# Autodesk Inventor assembly: AssemblyFullPrinter
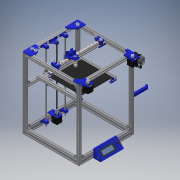
[picture p0: Inventor's stored thumbnail of the model, 180x180]
Saved by Autodesk Inventor 2018 (Build 220112000, 112)
## iProperties
Created: 2017-10-01
Part Number: AssemblyFullPrinter
Document SubType Name: Assembly
Designer: Jurjen
Author: Jurjen
## Documents named in this file (51)
- C:\Users\Jurjen\Documents\3D Printer\coreXY\Mechanical\AssemblyFullPrinter.iam
- C:\Users\Jurjen\Documents\3D Printer\coreXY\Mechanical\2020-350mm.ipt
- C:\Users\Jurjen\Documents\3D Printer\coreXY\Mechanical\2020-500mm.ipt
- C:\Users\Jurjen\Documents\3D Printer\coreXY\Mechanical\2020-corner-bracket.ipt
- C:\Users\Jurjen\Documents\3D Printer\coreXY\Mechanical\heated-bed.ipt
- C:\Users\Jurjen\Documents\3D Printer\coreXY\Mechanical\T8-lead-screw.ipt
- C:\Users\Jurjen\Documents\3D Printer\coreXY\Mechanical\motedis\GT2-Pulley-20-Teeth-5mm-Bore.ipt
- C:\Users\Jurjen\Documents\3D Printer\coreXY\Mechanical\motedis\Gt20.ipt
- C:\Users\Jurjen\Documents\3D Printer\coreXY\Mechanical\motedis\shaft-couple-flex.ipt
- C:\Users\Jurjen\Documents\3D Printer\coreXY\Mechanical\rod-8mm.ipt
- C:\Users\Jurjen\Documents\3D Printer\coreXY\Mechanical\2020-290mm.ipt
- C:\Users\Jurjen\Documents\3D Printer\coreXY\Mechanical\2020-240mm.ipt
- C:\Users\Jurjen\Documents\3D Printer\coreXY\Mechanical\T8x2mm lead screw.ipt
- C:\Users\Jurjen\Documents\3D Printer\coreXY\Mechanical\OldhamCouplerBottom.ipt
- C:\Users\Jurjen\Documents\3D Printer\coreXY\Mechanical\OldhamCouplerMiddle.ipt
- C:\Users\Jurjen\Documents\3D Printer\coreXY\Mechanical\OldhamCouplerTop.ipt
- C:\Users\Jurjen\Documents\3D Printer\coreXY\Mechanical\M5-nut.ipt
- C:\Users\Jurjen\Documents\3D Printer\coreXY\Mechanical\bracket-GT2-left.ipt
- C:\Users\Jurjen\Documents\3D Printer\coreXY\Mechanical\M5x30mm.ipt
- C:\Users\Jurjen\Documents\3D Printer\coreXY\Mechanical\mount-heated-bed.ipt
- C:\Users\Jurjen\Documents\3D Printer\coreXY\Mechanical\bracket-GT2-right.ipt
- C:\Users\Jurjen\Documents\3D Printer\coreXY\Mechanical\spool-holder.ipt
- C:\Users\Jurjen\Documents\3D Printer\coreXY\Mechanical\nema-17.ipt
- C:\Users\Jurjen\Documents\3D Printer\coreXY\Mechanical\nema17-mount-left.ipt
- C:\Users\Jurjen\Documents\3D Printer\coreXY\Mechanical\nema17-mount-right.ipt
- C:\Users\Jurjen\Documents\3D Printer\coreXY\Mechanical\LMF8LUU.ipt
- C:\Users\Jurjen\Documents\3D Printer\coreXY\Mechanical\MGN-12-rail.ipt
- C:\Users\Jurjen\Documents\3D Printer\coreXY\Mechanical\2020-320mm.ipt
- C:\Users\Jurjen\Documents\3D Printer\coreXY\Mechanical\x-carriage-2020.ipt
- C:\Users\Jurjen\Documents\3D Printer\coreXY\Mechanical\X-connector-left.ipt
- C:\Users\Jurjen\Documents\3D Printer\coreXY\Mechanical\X-connector-right.ipt
- C:\Users\Jurjen\Documents\3D Printer\coreXY\Mechanical\MGN-12-H-carriage.ipt
- C:\Users\Jurjen\Documents\3D Printer\coreXY\Mechanical\ED3V6.ipt
- C:\Users\Jurjen\Documents\3D Printer\coreXY\Mechanical\x-carriage.ipt
- C:\Users\Jurjen\Documents\3D Printer\coreXY\Mechanical\x-carriage-holder.ipt
- C:\Users\Jurjen\Documents\3D Printer\coreXY\Mechanical\holder-GT2-x-carriage-left.ipt
- C:\Users\Jurjen\Documents\3D Printer\coreXY\Mechanical\M5x35mm-crosshead.ipt
- C:\Users\Jurjen\Documents\3D Printer\coreXY\Mechanical\extruder\e3d titan.iam
- C:\Users\Jurjen\Documents\3D Printer\coreXY\Mechanical\mount-extruder.ipt
- C:\Users\Jurjen\Documents\3D Printer\coreXY\Mechanical\NylonSpacerM5x5mm.ipt
- C:\Users\Jurjen\Documents\3D Printer\coreXY\Mechanical\holder-GT2-x-carriage-right.ipt
- C:\Users\Jurjen\Documents\3D Printer\coreXY\Mechanical\holder-bearing-z-axis.ipt
- C:\Users\Jurjen\Documents\3D Printer\coreXY\Mechanical\2040-350mm.ipt
- C:\Users\Jurjen\Documents\3D Printer\coreXY\Mechanical\nema17-mount-bottom-z-axis-v2.ipt
- C:\Users\Jurjen\Documents\3D Printer\coreXY\Mechanical\ramps-1.4 2004-LCD.ipt
- C:\Users\Jurjen\Documents\3D Printer\coreXY\Mechanical\holder-LCD-screen.ipt
- C:\Users\Jurjen\Documents\3D Printer\coreXY\Mechanical\spring-25mm.ipt
- C:\Users\Jurjen\Documents\3D Printer\coreXY\Mechanical\M3x40mm.ipt
- C:\Users\Jurjen\Documents\3D Printer\coreXY\Mechanical\2040-360mm.ipt
- C:\Users\Jurjen\Documents\3D Printer\coreXY\Mechanical\SH8.ipt
- C:\Users\Jurjen\Documents\3D Printer\coreXY\Mechanical\holder-LMF8LUU-z-axis-v2.ipt
## Components (135 placed, 50 different names)
1. SH8:1 — Mate:601, Mate:602, Mate:603, Mate:604
2. SH8:2 — Mate:598, Mate:599, Mate:600, Mate:605
3. SH8:3 — Mate:606, Mate:607, Mate:611
4. SH8:4 — Mate:608, Mate:609, Mate:610
5. holder-LMF8LUU-z-axis-v2:1 — Mate:612, Mate:613, Mate:614, Mate:615, Mate:616, Mate:623
6. holder-LMF8LUU-z-axis-v2:2 — Mate:617, Mate:619, Mate:620, Mate:621, Mate:622
7. 2020-500mm:1 — Mate:1, Flush:2, Flush:14, Mate:90, Mate:92, Mate:93, Mate:94, Mate:166, Mate:168, Mate:287, Mate:288, Flush:54, Mate:359, Mate:360, Mate:459, Mate:471, Mate:472, Mate:473, Flush:92, Mate:552, Flush:107
8. 2020-500mm:2 — Mate:2, Flush:1, Flush:13, Flush:14, Mate:75, Mate:77, Mate:79, Mate:80, Mate:151, Mate:152, Mate:362, Mate:455, Mate:530, Flush:93, Mate:563, Flush:109, Flush:110
9. 2020-500mm:3 — Mate:8, Flush:12, Flush:13, Flush:15, Mate:82, Mate:83, Mate:136, Mate:138, Flush:67, Mate:367, Mate:456, Mate:501, Flush:85, Flush:86, Mate:516, Mate:517, Mate:562, Mate:585, Mate:591, Flush:115
10. 2020-500mm:4 — Mate:7, Flush:15, Flush:27, Mate:142, Mate:144, Mate:157, Mate:158, Mate:354, Flush:65, Mate:447, Mate:450, Mate:510, Mate:553, Flush:106, Mate:575, Flush:114, Mate:583, Mate:596
11. 2020-corner-bracket:38 — Mate:515, Mate:516, Mate:517
12. 2020-320mm:3 — Mate:353, Mate:354, Mate:355, Mate:356, Flush:65, Flush:66, Mate:357, Mate:358, Mate:368, Mate:369, Mate:373, Mate:374, Mate:388, Flush:73, Mate:446, Mate:448, Mate:460, Mate:461
13. 2020-320mm:4 — Flush:67, Mate:362, Mate:363, Mate:364, Flush:68, Mate:366, Flush:69, Mate:371, Mate:372, Mate:385, Mate:386, Mate:387, Flush:72, Mate:453, Mate:454, Mate:457, Mate:458
14. 2020-350mm:1 — Mate:1, Mate:2, Flush:1, Flush:2, Mate:19, Mate:23, Mate:76, Mate:95, Mate:294, Mate:303, Mate:304, Mate:307, Mate:308, Flush:66, Flush:68
15. 2020-350mm:4 — Mate:7, Mate:8, Flush:12, Mate:16, Mate:26, Flush:27, Mate:239, Mate:277, Mate:279, Flush:53, Mate:337, Flush:70, Mate:449, Mate:452, Mate:497, Mate:498, Mate:499, Mate:500, Flush:88, Flush:89, Mate:515, Mate:598, Mate:599, Mate:601, Mate:602
16. 2020-corner-bracket:1 — Mate:16, Mate:356, Mate:452
17. 2020-corner-bracket:2 — Mate:23, Mate:363, Mate:364
18. 2020-corner-bracket:3 — Mate:19, Mate:357, Mate:358
19. 2020-corner-bracket:4 — Mate:26, Mate:385, Mate:386
20. 2020-corner-bracket:10 — Mate:75, Mate:76, Mate:77
21. 2020-corner-bracket:13 — Mate:93, Mate:94, Mate:95, Mate:359
22. 2020-corner-bracket:33 — Mate:449, Mate:450
23. 2020-corner-bracket:34 — Mate:446, Mate:447, Mate:448
24. 2020-corner-bracket:35 — Mate:453, Mate:454, Mate:455
25. 2020-corner-bracket:36 — Mate:456, Mate:457, Mate:458
26. 2020-corner-bracket:37 — Mate:459, Mate:460, Mate:461
27. 2040-360mm:1 — Mate:552, Mate:553, Flush:106, Flush:107, Mate:554, Mate:555, Mate:558, Mate:559, Flush:108
28. 2040-360mm:2 — Mate:562, Mate:563, Flush:109, Flush:110, Mate:564, Mate:565, Mate:567, Flush:111, Mate:571, Flush:115
29. ramps-1.4 2004-LCD:1 — Flush:96, Mate:535, Mate:536
30. holder-LCD-screen:1 — Mate:534, Flush:95, Flush:96, Mate:535, Mate:536
31. 2040-350mm:1 — Mate:501, Flush:85, Flush:86, Mate:502, Mate:503, Mate:509, Flush:87, Mate:524, Mate:525, Mate:606, Mate:607, Mate:609, Mate:610
32. 2040-350mm:2 — Mate:526, Mate:527, Mate:528, Mate:529, Flush:92, Mate:530, Flush:93, Mate:534, Flush:95
33. 2020-corner-bracket:5 — Mate:503, Mate:559, Mate:560
34. 2020-corner-bracket:6 — Mate:502, Mate:570, Mate:571
35. 2020-corner-bracket:7 — Mate:528, Mate:567, Mate:569
36. 2020-corner-bracket:8 — Mate:529, Mate:558, Mate:561
37. 2020-corner-bracket:9 — Mate:79, Mate:80, Mate:526
38. 2020-corner-bracket:11 — Mate:82, Mate:83, Mate:565
39. 2020-corner-bracket:12 — Mate:90, Mate:92, Mate:527
40. 2020-corner-bracket:23 — Mate:151, Mate:152, Mate:564
41. 2020-corner-bracket:25 — Mate:157, Mate:158, Mate:555
42. 2020-corner-bracket:28 — Mate:166, Mate:168, Mate:554
43. 2020-corner-bracket:19 — Mate:136, Mate:138, Mate:524
44. 2020-corner-bracket:20 — Mate:142, Mate:144, Mate:525
45. 2020-corner-bracket:41 — Mate:548, Mate:549, Mate:550
46. 2020-corner-bracket:42 — Mate:545, Mate:546, Mate:547
47. spring-25mm:1 — Mate:537, Flush:98
48. spring-25mm:2 — Mate:538, Flush:100
49. spring-25mm:3 — Mate:539, Flush:97
50. spring-25mm:4 — Mate:540, Flush:99
51. 2020-corner-bracket:14 — Mate:122, Mate:123, Mate:124
52. 2020-corner-bracket:15 — Mate:119, Mate:120, Mate:121, Flush:49
53. nema17-mount-bottom-z-axis-v2:1 — Mate:506, Mate:507, Mate:508, Mate:509, Flush:87, Mate:510
54. holder-bearing-z-axis:1 — Mate:498, Mate:499, Mate:500, Flush:89, Mate:604, Mate:605
55. shaft-couple-flex:1 — Mate:59, Mate:114, Mate:293
56. LMF8LUU:1 — Mate:313, Mate:612, Mate:613, Mate:614
57. LMF8LUU:2 — Mate:314, Mate:620, Mate:621, Mate:622
58. T8-lead-screw:1 — Mate:59, Mate:114, Mate:115, Mate:116, Mate:117, Mate:118, Mate:315
59. nema-17:1 — Mate:293, Mate:315, Mate:506, Mate:507, Mate:508
60. rod-8mm:1 — Mate:314, Mate:600, Mate:611
61. rod-8mm:2 — Mate:313, Mate:603, Mate:608
62. heated-bed:1 — Mate:267, Mate:269, Mate:272, Mate:275, Mate:276, Mate:541, Flush:101, Flush:102, Mate:542, Mate:543, Flush:103, Flush:104, Mate:544
63. 2020-290mm:1 — Mate:109, Flush:45, Flush:46, Mate:123, Mate:265, Mate:266, Flush:52, Mate:270, Mate:271, Mate:545
64. 2020-290mm:2 — Mate:107, Flush:45, Flush:47, Mate:119, Flush:49, Mate:263, Mate:264, Flush:51, Mate:273, Mate:274, Mate:549
65. 2020-240mm:1 — Mate:103, Mate:104, Mate:105, Mate:107, Mate:109, Flush:46, Flush:47, Mate:110, Mate:120, Mate:121, Mate:122, Mate:124, Flush:88, Mate:546, Mate:547, Mate:548, Mate:550, Mate:615, Mate:616, Mate:617, Mate:619, Mate:623
66. mount-heated-bed:1 — Mate:263, Mate:264, Flush:51, Mate:267, Mate:276, Mate:537, Flush:98
67. mount-heated-bed:2 — Mate:265, Mate:266, Flush:52, Mate:269, Mate:538, Flush:100
68. mount-heated-bed:3 — Mate:270, Mate:271, Mate:272, Mate:540, Flush:99
69. mount-heated-bed:4 — Mate:273, Mate:274, Mate:275, Mate:539, Flush:97
70. M3x40mm:1 — Mate:541, Flush:101
71. M3x40mm:2 — Flush:102, Mate:542
72. M3x40mm:3 — Mate:543, Flush:103
73. M3x40mm:4 — Flush:104, Mate:544
74. Gt20:9 — Mate:486, Mate:488, Mate:489, Flush:83
75. Gt20:10 — Mate:485, Mate:496, Flush:84
76. NylonSpacerM5x5mm:3 — Mate:490, Mate:491
77. NylonSpacerM5x5mm:4 — Mate:487, Mate:489, Mate:491
78. M5-nut:9 — Mate:494, Mate:495
79. M5-nut:10 — Mate:492, Mate:493
80. M5x35mm-crosshead:3 — Mate:484, Mate:486, Mate:487, Mate:488, Mate:490, Mate:492
81. M5x35mm-crosshead:4 — Mate:483, Mate:485, Mate:494, Mate:496
82. holder-GT2-x-carriage-right:1 — Mate:480, Mate:481, Mate:482, Mate:483, Mate:484, Mate:493, Mate:495
83. NylonSpacerM5x5mm:2 — Mate:476, Mate:477
84. NylonSpacerM5x5mm:1 — Mate:474, Mate:475, Mate:477
85. Gt20:7 — Mate:424, Mate:433, Flush:76
86. Gt20:8 — Mate:423, Mate:427, Flush:77, Mate:475
87. MGN-12-rail:2 — Mate:373, Mate:374, Mate:388, Mate:394, Mate:395, Flush:73
88. MGN-12-rail:3 — Mate:371, Mate:372, Mate:387, Mate:392, Mate:393, Flush:72
89. MGN-12-H-carriage:1 — Mate:392, Mate:393, Mate:399, Mate:415
90. MGN-12-H-carriage:3 — Mate:394, Mate:395, Mate:396, Mate:397, Mate:398
91. GT2-Pulley-20-Teeth-5mm-Bore:2 — Mate:312, Flush:75, Flush:84
92. GT2-Pulley-20-Teeth-5mm-Bore:1 — Mate:297, Flush:56
93. bracket-GT2-right:1 — Mate:277, Mate:279, Mate:280, Mate:281, Mate:283, Mate:284, Mate:285, Mate:286, Flush:53, Mate:353, Mate:355
94. Gt20:5 — Mate:240, Mate:241, Flush:56, Mate:419, Flush:77
95. Gt20:6 — Mate:242, Mate:243, Mate:262, Flush:76
96. M5-nut:6 — Mate:260, Mate:283
97. bracket-GT2-left:1 — Mate:237, Mate:238, Mate:239, Mate:245, Mate:247, Mate:262, Mate:366, Mate:367, Flush:70, Mate:419
98. M5-nut:3 — Mate:244, Mate:245
99. M5-nut:5 — Mate:246, Mate:247
100. M5x30mm:1 — Mate:237, Mate:240, Mate:241, Mate:244
101. M5x30mm:2 — Mate:238, Mate:242, Mate:243, Mate:246
102. M5x30mm:3 — Mate:254, Mate:256, Mate:260, Mate:281
103. M5x30mm:4 — Mate:255, Mate:257, Mate:258, Mate:280
104. Gt20:2 — Mate:254, Mate:256, Mate:286, Flush:75
105. Gt20:4 — Mate:255, Mate:257, Mate:285, Flush:83
106. M5-nut:2 — Mate:258, Mate:284
107. nema-17:2 — Mate:297, Mate:298, Mate:299, Mate:300, Flush:57
108. nema-17:3 — Mate:309, Mate:310, Flush:58, Mate:311, Mate:312
109. nema17-mount-left:1 — Mate:294, Mate:298, Mate:299, Mate:300, Flush:57, Mate:303, Mate:304, Flush:69
110. nema17-mount-right:1 — Mate:307, Mate:308, Mate:309, Mate:310, Flush:58, Mate:311, Mate:360, Mate:368, Mate:369
111. spool-holder:1 — Mate:287, Mate:288, Flush:54
112. e3d titan:1 [sub-assembly] — Mate:465, Mate:466, Mate:470
113. mount-extruder:1 — Mate:465, Mate:466, Mate:467, Mate:468, Mate:469, Mate:470, Mate:471, Mate:472, Mate:473
114. nema-17:4 — Mate:467, Mate:468, Mate:469
115. 2020-350mm:12 — Mate:575, Flush:114, Mate:577, Mate:581, Mate:587, Mate:597
116. 2020-corner-bracket:44 — Mate:577, Mate:583, Mate:596
117. 2020-corner-bracket:45 — Mate:587, Mate:597
118. 2020-corner-bracket:49 — Mate:581, Mate:585, Mate:591
119. T8x2mm lead screw:1 — Mate:100, Mate:118
120. OldhamCouplerBottom:1 — Mate:99, Flush:43, Mate:100, Mate:117
121. OldhamCouplerMiddle:1 — Mate:99, Flush:43, Flush:44, Mate:102, Mate:115
122. OldhamCouplerTop:1 — Flush:44, Mate:102, Mate:103, Mate:104, Mate:105, Mate:110, Mate:116, Mate:337
123. MGN-12-rail:1 — Mate:381, Mate:389, Mate:390, Mate:391, Flush:71
124. x-carriage-2020:1 — Mate:377, Mate:381, Mate:384, Mate:389, Flush:71, Mate:409, Mate:410, Mate:411, Mate:421, Mate:422, Mate:432, Mate:480, Mate:481, Mate:482, Mate:497
125. X-connector-left:1 — Mate:377, Mate:396, Mate:397, Mate:398, Mate:410, Mate:411
126. X-connector-right:1 — Mate:384, Mate:399, Mate:409, Mate:415
127. MGN-12-H-carriage:2 — Mate:390, Mate:391, Mate:402, Mate:403, Mate:404
128. x-carriage-holder:1 — Mate:408, Mate:478, Mate:479
129. x-carriage:1 — Mate:402, Mate:403, Mate:404, Mate:405, Mate:408, Flush:74, Mate:478, Mate:479, Mate:514
130. holder-GT2-x-carriage-left:1 — Mate:421, Mate:422, Mate:425, Mate:426, Mate:429, Mate:431, Mate:432, Mate:514
131. M5-nut:7 — Mate:428, Mate:429
132. M5x35mm-crosshead:1 — Mate:423, Mate:426, Mate:427, Mate:428, Mate:474, Mate:476
133. M5-nut:8 — Mate:430, Mate:431
134. M5x35mm-crosshead:2 — Mate:424, Mate:425, Mate:430, Mate:433
135. ED3V6:1 — Mate:405, Flush:74
## Relationships (367: Mate 307, Flush 60)
- Mate:1: 2020-500mm:1 ↔ 2020-350mm:1
- Mate:2: 2020-500mm:2 ↔ 2020-350mm:1
- Flush:1: 2020-500mm:2 ↔ 2020-350mm:1
- Flush:2: 2020-500mm:1 ↔ 2020-350mm:1
- Mate:7: 2020-500mm:4 ↔ 2020-350mm:4
- Mate:8: 2020-500mm:3 ↔ 2020-350mm:4
- Flush:12: 2020-500mm:3 ↔ 2020-350mm:4
- Flush:13: 2020-500mm:2 ↔ 2020-500mm:3
- Flush:14: 2020-500mm:1 ↔ 2020-500mm:2
- Flush:15: 2020-500mm:3 ↔ 2020-500mm:4
- Mate:16: 2020-350mm:4 ↔ 2020-corner-bracket:1
- Mate:19: 2020-350mm:1 ↔ 2020-corner-bracket:3
- Mate:23: 2020-350mm:1 ↔ 2020-corner-bracket:2
- Mate:26: 2020-350mm:4 ↔ 2020-corner-bracket:4
- Flush:27: 2020-500mm:4 ↔ 2020-350mm:4
- Mate:59 (-8 mm): shaft-couple-flex:1 ↔ T8-lead-screw:1
- Mate:75: 2020-500mm:2 ↔ 2020-corner-bracket:10
- Mate:76: 2020-350mm:1 ↔ 2020-corner-bracket:10
- Mate:77: 2020-500mm:2 ↔ 2020-corner-bracket:10
- Mate:79: 2020-500mm:2 ↔ 2020-corner-bracket:9
- Mate:80: 2020-500mm:2 ↔ 2020-corner-bracket:9
- Mate:82: 2020-500mm:3 ↔ 2020-corner-bracket:11
- Mate:83: 2020-500mm:3 ↔ 2020-corner-bracket:11
- Mate:90: 2020-500mm:1 ↔ 2020-corner-bracket:12
- Mate:92: 2020-500mm:1 ↔ 2020-corner-bracket:12
- Mate:93: 2020-500mm:1 ↔ 2020-corner-bracket:13
- Mate:94: 2020-500mm:1 ↔ 2020-corner-bracket:13
- Mate:95: 2020-350mm:1 ↔ 2020-corner-bracket:13
- Mate:99: OldhamCouplerBottom:1 ↔ OldhamCouplerMiddle:1
- Flush:43: OldhamCouplerBottom:1 ↔ OldhamCouplerMiddle:1
- Mate:100: T8x2mm lead screw:1 ↔ OldhamCouplerBottom:1
- Flush:44: OldhamCouplerMiddle:1 ↔ OldhamCouplerTop:1
- Mate:102: OldhamCouplerMiddle:1 ↔ OldhamCouplerTop:1
- Mate:103: 2020-240mm:1 ↔ OldhamCouplerTop:1
- Mate:104: 2020-240mm:1 ↔ OldhamCouplerTop:1
- Mate:105: 2020-240mm:1 ↔ OldhamCouplerTop:1
- Mate:107: 2020-290mm:2 ↔ 2020-240mm:1
- Mate:109: 2020-290mm:1 ↔ 2020-240mm:1
- Flush:45: 2020-290mm:1 ↔ 2020-290mm:2
- Flush:46: 2020-290mm:1 ↔ 2020-240mm:1
- Flush:47: 2020-290mm:2 ↔ 2020-240mm:1
- Mate:110: 2020-240mm:1 ↔ OldhamCouplerTop:1
- Mate:114: shaft-couple-flex:1 ↔ T8-lead-screw:1
- Mate:115: T8-lead-screw:1 ↔ OldhamCouplerMiddle:1
- Mate:116: T8-lead-screw:1 ↔ OldhamCouplerTop:1
- Mate:117: T8-lead-screw:1 ↔ OldhamCouplerBottom:1
- Mate:118: T8-lead-screw:1 ↔ T8x2mm lead screw:1
- Mate:119: 2020-corner-bracket:15 ↔ 2020-290mm:2
- Mate:120: 2020-corner-bracket:15 ↔ 2020-240mm:1
- Mate:121: 2020-corner-bracket:15 ↔ 2020-240mm:1
- Flush:49: 2020-corner-bracket:15 ↔ 2020-290mm:2
- Mate:122: 2020-corner-bracket:14 ↔ 2020-240mm:1
- Mate:123: 2020-corner-bracket:14 ↔ 2020-290mm:1
- Mate:124: 2020-corner-bracket:14 ↔ 2020-240mm:1
- Mate:136: 2020-500mm:3 ↔ 2020-corner-bracket:19
- Mate:138: 2020-500mm:3 ↔ 2020-corner-bracket:19
- Mate:142: 2020-500mm:4 ↔ 2020-corner-bracket:20
- Mate:144: 2020-500mm:4 ↔ 2020-corner-bracket:20
- Mate:151: 2020-500mm:2 ↔ 2020-corner-bracket:23
- Mate:152: 2020-500mm:2 ↔ 2020-corner-bracket:23
- Mate:157: 2020-500mm:4 ↔ 2020-corner-bracket:25
- Mate:158: 2020-500mm:4 ↔ 2020-corner-bracket:25
- Mate:166: 2020-500mm:1 ↔ 2020-corner-bracket:28
- Mate:168: 2020-500mm:1 ↔ 2020-corner-bracket:28
- Mate:237: bracket-GT2-left:1 ↔ M5x30mm:1
- Mate:238: bracket-GT2-left:1 ↔ M5x30mm:2
- Mate:239: 2020-350mm:4 ↔ bracket-GT2-left:1
- Mate:240: Gt20:5 ↔ M5x30mm:1
- Mate:241: Gt20:5 ↔ M5x30mm:1
- Mate:242: Gt20:6 ↔ M5x30mm:2
- Mate:243: Gt20:6 ↔ M5x30mm:2
- Mate:244: M5-nut:3 ↔ M5x30mm:1
- Mate:245: bracket-GT2-left:1 ↔ M5-nut:3
- Mate:246: M5-nut:5 ↔ M5x30mm:2
- Mate:247: bracket-GT2-left:1 ↔ M5-nut:5
- Mate:254: M5x30mm:3 ↔ Gt20:2
- Mate:255: M5x30mm:4 ↔ Gt20:4
- Mate:256: M5x30mm:3 ↔ Gt20:2
- Mate:257: M5x30mm:4 ↔ Gt20:4
- Mate:258: M5x30mm:4 ↔ M5-nut:2
- Mate:260: M5-nut:6 ↔ M5x30mm:3
- Mate:262: Gt20:6 ↔ bracket-GT2-left:1
- Mate:263: 2020-290mm:2 ↔ mount-heated-bed:1
- Mate:264: 2020-290mm:2 ↔ mount-heated-bed:1
- Flush:51: 2020-290mm:2 ↔ mount-heated-bed:1
- Mate:265: 2020-290mm:1 ↔ mount-heated-bed:2
- Mate:266: 2020-290mm:1 ↔ mount-heated-bed:2
- Flush:52: 2020-290mm:1 ↔ mount-heated-bed:2
- Mate:267: heated-bed:1 ↔ mount-heated-bed:1
- Mate:269: heated-bed:1 ↔ mount-heated-bed:2
- Mate:270: 2020-290mm:1 ↔ mount-heated-bed:3
- Mate:271: 2020-290mm:1 ↔ mount-heated-bed:3
- Mate:272: heated-bed:1 ↔ mount-heated-bed:3
- Mate:273: 2020-290mm:2 ↔ mount-heated-bed:4
- Mate:274: 2020-290mm:2 ↔ mount-heated-bed:4
- Mate:275: heated-bed:1 ↔ mount-heated-bed:4
- Mate:276 (25 mm): heated-bed:1 ↔ mount-heated-bed:1
- Mate:277: 2020-350mm:4 ↔ bracket-GT2-right:1
- Mate:279: 2020-350mm:4 ↔ bracket-GT2-right:1
- Mate:280: bracket-GT2-right:1 ↔ M5x30mm:4
- Mate:281: bracket-GT2-right:1 ↔ M5x30mm:3
- Mate:283: bracket-GT2-right:1 ↔ M5-nut:6
- Mate:284: bracket-GT2-right:1 ↔ M5-nut:2
- Mate:285: bracket-GT2-right:1 ↔ Gt20:4
- Mate:286: bracket-GT2-right:1 ↔ Gt20:2
- Flush:53: 2020-350mm:4 ↔ bracket-GT2-right:1
- Mate:287: 2020-500mm:1 ↔ spool-holder:1
- Mate:288: 2020-500mm:1 ↔ spool-holder:1
- Flush:54: 2020-500mm:1 ↔ spool-holder:1
- Mate:293 (-8 mm): shaft-couple-flex:1 ↔ nema-17:1
- Mate:294: 2020-350mm:1 ↔ nema17-mount-left:1
- Mate:297: GT2-Pulley-20-Teeth-5mm-Bore:1 ↔ nema-17:2
- Flush:56: GT2-Pulley-20-Teeth-5mm-Bore:1 ↔ Gt20:5
- Mate:298: nema-17:2 ↔ nema17-mount-left:1
- Mate:299: nema-17:2 ↔ nema17-mount-left:1
- Mate:300: nema-17:2 ↔ nema17-mount-left:1
- Flush:57: nema-17:2 ↔ nema17-mount-left:1
- Mate:303: 2020-350mm:1 ↔ nema17-mount-left:1
- Mate:304: 2020-350mm:1 ↔ nema17-mount-left:1
- Mate:307: 2020-350mm:1 ↔ nema17-mount-right:1
- Mate:308: 2020-350mm:1 ↔ nema17-mount-right:1
- Mate:309: nema-17:3 ↔ nema17-mount-right:1
- Mate:310: nema-17:3 ↔ nema17-mount-right:1
- Flush:58: nema-17:3 ↔ nema17-mount-right:1
- Mate:311: nema-17:3 ↔ nema17-mount-right:1
- Mate:312: GT2-Pulley-20-Teeth-5mm-Bore:2 ↔ nema-17:3
- Mate:313: LMF8LUU:1 ↔ rod-8mm:2
- Mate:314: LMF8LUU:2 ↔ rod-8mm:1
- Mate:315: T8-lead-screw:1 ↔ nema-17:1
- Mate:337: 2020-350mm:4 ↔ OldhamCouplerTop:1
- Mate:353: 2020-320mm:3 ↔ bracket-GT2-right:1
- Mate:354: 2020-500mm:4 ↔ 2020-320mm:3
- Mate:355: 2020-320mm:3 ↔ bracket-GT2-right:1
- Mate:356: 2020-320mm:3 ↔ 2020-corner-bracket:1
- Flush:65: 2020-500mm:4 ↔ 2020-320mm:3
- Flush:66: 2020-320mm:3 ↔ 2020-350mm:1
- Mate:357: 2020-320mm:3 ↔ 2020-corner-bracket:3
- Mate:358: 2020-320mm:3 ↔ 2020-corner-bracket:3
- Mate:359: 2020-500mm:1 ↔ 2020-corner-bracket:13
- Mate:360: 2020-500mm:1 ↔ nema17-mount-right:1
- Flush:67: 2020-500mm:3 ↔ 2020-320mm:4
- Mate:362: 2020-500mm:2 ↔ 2020-320mm:4
- Mate:363: 2020-320mm:4 ↔ 2020-corner-bracket:2
- Mate:364: 2020-320mm:4 ↔ 2020-corner-bracket:2
- Flush:68: 2020-320mm:4 ↔ 2020-350mm:1
- Mate:366: 2020-320mm:4 ↔ bracket-GT2-left:1
- Mate:367: 2020-500mm:3 ↔ bracket-GT2-left:1
- Mate:368: 2020-320mm:3 ↔ nema17-mount-right:1
- Mate:369: 2020-320mm:3 ↔ nema17-mount-right:1
- Flush:69: 2020-320mm:4 ↔ nema17-mount-left:1
- Mate:371: 2020-320mm:4 ↔ MGN-12-rail:3
- Mate:372: 2020-320mm:4 ↔ MGN-12-rail:3
- Mate:373: 2020-320mm:3 ↔ MGN-12-rail:2
- Mate:374: 2020-320mm:3 ↔ MGN-12-rail:2
- Flush:70: 2020-350mm:4 ↔ bracket-GT2-left:1
- Mate:377: x-carriage-2020:1 ↔ X-connector-left:1
- Mate:381: MGN-12-rail:1 ↔ x-carriage-2020:1
- Mate:384: x-carriage-2020:1 ↔ X-connector-right:1
- Mate:385: 2020-320mm:4 ↔ 2020-corner-bracket:4
- Mate:386: 2020-320mm:4 ↔ 2020-corner-bracket:4
- Mate:387: 2020-320mm:4 ↔ MGN-12-rail:3
- Mate:388: 2020-320mm:3 ↔ MGN-12-rail:2
- Mate:389: MGN-12-rail:1 ↔ x-carriage-2020:1
- Mate:390: MGN-12-rail:1 ↔ MGN-12-H-carriage:2
- Mate:391: MGN-12-rail:1 ↔ MGN-12-H-carriage:2
- Mate:392: MGN-12-rail:3 ↔ MGN-12-H-carriage:1
- Mate:393: MGN-12-rail:3 ↔ MGN-12-H-carriage:1
- Mate:394: MGN-12-rail:2 ↔ MGN-12-H-carriage:3
- Mate:395: MGN-12-rail:2 ↔ MGN-12-H-carriage:3
- Mate:396: MGN-12-H-carriage:3 ↔ X-connector-left:1
- Mate:397: MGN-12-H-carriage:3 ↔ X-connector-left:1
- Mate:398: MGN-12-H-carriage:3 ↔ X-connector-left:1
- Mate:399: MGN-12-H-carriage:1 ↔ X-connector-right:1
- Flush:71: MGN-12-rail:1 ↔ x-carriage-2020:1
- Flush:72: 2020-320mm:4 ↔ MGN-12-rail:3
- Flush:73: 2020-320mm:3 ↔ MGN-12-rail:2
- Mate:402: MGN-12-H-carriage:2 ↔ x-carriage:1
- Mate:403: MGN-12-H-carriage:2 ↔ x-carriage:1
- Mate:404: MGN-12-H-carriage:2 ↔ x-carriage:1
- Mate:405: x-carriage:1 ↔ ED3V6:1
- Mate:408: x-carriage-holder:1 ↔ x-carriage:1
- Flush:74: x-carriage:1 ↔ ED3V6:1
- Flush:75: GT2-Pulley-20-Teeth-5mm-Bore:2 ↔ Gt20:2
- Mate:409: x-carriage-2020:1 ↔ X-connector-right:1
- Mate:410: x-carriage-2020:1 ↔ X-connector-left:1
- Mate:411 (-25 mm): x-carriage-2020:1 ↔ X-connector-left:1
- Mate:415: MGN-12-H-carriage:1 ↔ X-connector-right:1
- Mate:419: Gt20:5 ↔ bracket-GT2-left:1
- Mate:421: x-carriage-2020:1 ↔ holder-GT2-x-carriage-left:1
- Mate:422: x-carriage-2020:1 ↔ holder-GT2-x-carriage-left:1
- Mate:423: Gt20:8 ↔ M5x35mm-crosshead:1
- Mate:424: Gt20:7 ↔ M5x35mm-crosshead:2
- Mate:425: holder-GT2-x-carriage-left:1 ↔ M5x35mm-crosshead:2
- Mate:426: holder-GT2-x-carriage-left:1 ↔ M5x35mm-crosshead:1
- Mate:427: Gt20:8 ↔ M5x35mm-crosshead:1
- Mate:428: M5-nut:7 ↔ M5x35mm-crosshead:1
- Mate:429: holder-GT2-x-carriage-left:1 ↔ M5-nut:7
- Mate:430: M5-nut:8 ↔ M5x35mm-crosshead:2
- Mate:431: holder-GT2-x-carriage-left:1 ↔ M5-nut:8
- Mate:432: x-carriage-2020:1 ↔ holder-GT2-x-carriage-left:1
- Mate:433: Gt20:7 ↔ M5x35mm-crosshead:2
- Flush:76: Gt20:7 ↔ Gt20:6
- Flush:77: Gt20:8 ↔ Gt20:5
- Mate:446: 2020-320mm:3 ↔ 2020-corner-bracket:34
- Mate:447: 2020-500mm:4 ↔ 2020-corner-bracket:34
- Mate:448: 2020-320mm:3 ↔ 2020-corner-bracket:34
- Mate:449: 2020-350mm:4 ↔ 2020-corner-bracket:33
- Mate:450: 2020-500mm:4 ↔ 2020-corner-bracket:33
- Mate:452: 2020-350mm:4 ↔ 2020-corner-bracket:1
- Mate:453: 2020-320mm:4 ↔ 2020-corner-bracket:35
- Mate:454: 2020-320mm:4 ↔ 2020-corner-bracket:35
- Mate:455: 2020-500mm:2 ↔ 2020-corner-bracket:35
- Mate:456: 2020-500mm:3 ↔ 2020-corner-bracket:36
- Mate:457: 2020-320mm:4 ↔ 2020-corner-bracket:36
- Mate:458: 2020-320mm:4 ↔ 2020-corner-bracket:36
- Mate:459: 2020-500mm:1 ↔ 2020-corner-bracket:37
- Mate:460: 2020-320mm:3 ↔ 2020-corner-bracket:37
- Mate:461: 2020-320mm:3 ↔ 2020-corner-bracket:37
- Mate:465: e3d titan:1 ↔ mount-extruder:1
- Mate:466: e3d titan:1 ↔ mount-extruder:1
- Mate:467: mount-extruder:1 ↔ nema-17:4
- Mate:468: mount-extruder:1 ↔ nema-17:4
- Mate:469: mount-extruder:1 ↔ nema-17:4
- Mate:470: e3d titan:1 ↔ mount-extruder:1
- Mate:471: 2020-500mm:1 ↔ mount-extruder:1
- Mate:472: 2020-500mm:1 ↔ mount-extruder:1
- Mate:473: 2020-500mm:1 ↔ mount-extruder:1
- Mate:474: NylonSpacerM5x5mm:1 ↔ M5x35mm-crosshead:1
- Mate:475: NylonSpacerM5x5mm:1 ↔ Gt20:8
- Mate:476: NylonSpacerM5x5mm:2 ↔ M5x35mm-crosshead:1
- Mate:477: NylonSpacerM5x5mm:2 ↔ NylonSpacerM5x5mm:1
- Mate:478: x-carriage-holder:1 ↔ x-carriage:1
- Mate:479: x-carriage-holder:1 ↔ x-carriage:1
- Mate:480: holder-GT2-x-carriage-right:1 ↔ x-carriage-2020:1
- Mate:481: holder-GT2-x-carriage-right:1 ↔ x-carriage-2020:1
- Mate:482: holder-GT2-x-carriage-right:1 ↔ x-carriage-2020:1
- Mate:483: M5x35mm-crosshead:4 ↔ holder-GT2-x-carriage-right:1
- Mate:484: M5x35mm-crosshead:3 ↔ holder-GT2-x-carriage-right:1
- Mate:485: Gt20:10 ↔ M5x35mm-crosshead:4
- Mate:486: Gt20:9 ↔ M5x35mm-crosshead:3
- Mate:487: NylonSpacerM5x5mm:4 ↔ M5x35mm-crosshead:3
- Mate:488: Gt20:9 ↔ M5x35mm-crosshead:3
- Mate:489: Gt20:9 ↔ NylonSpacerM5x5mm:4
- Mate:490: NylonSpacerM5x5mm:3 ↔ M5x35mm-crosshead:3
- Mate:491: NylonSpacerM5x5mm:3 ↔ NylonSpacerM5x5mm:4
- Mate:492: M5-nut:10 ↔ M5x35mm-crosshead:3
- Mate:493: M5-nut:10 ↔ holder-GT2-x-carriage-right:1
- Flush:83: Gt20:9 ↔ Gt20:4
- Mate:494: M5-nut:9 ↔ M5x35mm-crosshead:4
- Mate:495: M5-nut:9 ↔ holder-GT2-x-carriage-right:1
- Mate:496: Gt20:10 ↔ M5x35mm-crosshead:4
- Flush:84: Gt20:10 ↔ GT2-Pulley-20-Teeth-5mm-Bore:2
- Mate:497: 2020-350mm:4 ↔ x-carriage-2020:1
- Mate:498: 2020-350mm:4 ↔ holder-bearing-z-axis:1
- Mate:499: 2020-350mm:4 ↔ holder-bearing-z-axis:1
- Mate:500: 2020-350mm:4 ↔ holder-bearing-z-axis:1
- Mate:501: 2020-500mm:3 ↔ 2040-350mm:1
- Flush:85: 2020-500mm:3 ↔ 2040-350mm:1
- Flush:86: 2020-500mm:3 ↔ 2040-350mm:1
- Mate:502: 2040-350mm:1 ↔ 2020-corner-bracket:6
- Mate:503: 2040-350mm:1 ↔ 2020-corner-bracket:5
- Mate:506: nema17-mount-bottom-z-axis-v2:1 ↔ nema-17:1
- Mate:507: nema17-mount-bottom-z-axis-v2:1 ↔ nema-17:1
- Mate:508: nema17-mount-bottom-z-axis-v2:1 ↔ nema-17:1
- Mate:509: 2040-350mm:1 ↔ nema17-mount-bottom-z-axis-v2:1
- Flush:87: 2040-350mm:1 ↔ nema17-mount-bottom-z-axis-v2:1
- Mate:510 (155 mm): 2020-500mm:4 ↔ nema17-mount-bottom-z-axis-v2:1
- Flush:88: 2020-350mm:4 ↔ 2020-240mm:1
- Flush:89: 2020-350mm:4 ↔ holder-bearing-z-axis:1
- Mate:514: x-carriage:1 ↔ holder-GT2-x-carriage-left:1
- Mate:515: 2020-corner-bracket:38 ↔ 2020-350mm:4
- Mate:516: 2020-500mm:3 ↔ 2020-corner-bracket:38
- Mate:517: 2020-500mm:3 ↔ 2020-corner-bracket:38
- Mate:524: 2040-350mm:1 ↔ 2020-corner-bracket:19
- Mate:525: 2040-350mm:1 ↔ 2020-corner-bracket:20
- Mate:526: 2040-350mm:2 ↔ 2020-corner-bracket:9
- Mate:527: 2040-350mm:2 ↔ 2020-corner-bracket:12
- Mate:528: 2040-350mm:2 ↔ 2020-corner-bracket:7
- Mate:529: 2040-350mm:2 ↔ 2020-corner-bracket:8
- Flush:92: 2020-500mm:1 ↔ 2040-350mm:2
- Mate:530: 2020-500mm:2 ↔ 2040-350mm:2
- Flush:93: 2020-500mm:2 ↔ 2040-350mm:2
- Mate:534: holder-LCD-screen:1 ↔ 2040-350mm:2
- Flush:95: holder-LCD-screen:1 ↔ 2040-350mm:2
- Flush:96 (-2 mm): ramps-1.4 2004-LCD:1 ↔ holder-LCD-screen:1
- Mate:535: ramps-1.4 2004-LCD:1 ↔ holder-LCD-screen:1
- Mate:536: ramps-1.4 2004-LCD:1 ↔ holder-LCD-screen:1
- Mate:537: spring-25mm:1 ↔ mount-heated-bed:1
- Mate:538: spring-25mm:2 ↔ mount-heated-bed:2
- Mate:539: spring-25mm:3 ↔ mount-heated-bed:4
- Flush:97: spring-25mm:3 ↔ mount-heated-bed:4
- Flush:98: spring-25mm:1 ↔ mount-heated-bed:1
- Mate:540: spring-25mm:4 ↔ mount-heated-bed:3
- Flush:99: spring-25mm:4 ↔ mount-heated-bed:3
- Flush:100: spring-25mm:2 ↔ mount-heated-bed:2
- Mate:541: heated-bed:1 ↔ M3x40mm:1
- Flush:101: heated-bed:1 ↔ M3x40mm:1
- Flush:102: heated-bed:1 ↔ M3x40mm:2
- Mate:542: heated-bed:1 ↔ M3x40mm:2
- Mate:543: heated-bed:1 ↔ M3x40mm:3
- Flush:103: heated-bed:1 ↔ M3x40mm:3
- Flush:104: heated-bed:1 ↔ M3x40mm:4
- Mate:544: heated-bed:1 ↔ M3x40mm:4
- Mate:545: 2020-corner-bracket:42 ↔ 2020-290mm:1
- Mate:546: 2020-corner-bracket:42 ↔ 2020-240mm:1
- Mate:547: 2020-corner-bracket:42 ↔ 2020-240mm:1
- Mate:548: 2020-corner-bracket:41 ↔ 2020-240mm:1
- Mate:549: 2020-corner-bracket:41 ↔ 2020-290mm:2
- Mate:550: 2020-corner-bracket:41 ↔ 2020-240mm:1
- Mate:552: 2020-500mm:1 ↔ 2040-360mm:1
- Mate:553: 2020-500mm:4 ↔ 2040-360mm:1
- Flush:106: 2020-500mm:4 ↔ 2040-360mm:1
- Flush:107: 2020-500mm:1 ↔ 2040-360mm:1
- Mate:554: 2040-360mm:1 ↔ 2020-corner-bracket:28
- Mate:555: 2040-360mm:1 ↔ 2020-corner-bracket:25
- Mate:558: 2040-360mm:1 ↔ 2020-corner-bracket:8
- Mate:559: 2040-360mm:1 ↔ 2020-corner-bracket:5
- Flush:108 (-10 mm): 2040-360mm:1
- Mate:560: 2020-corner-bracket:5
- Mate:561: 2020-corner-bracket:8
- Mate:562: 2020-500mm:3 ↔ 2040-360mm:2
- Mate:563: 2020-500mm:2 ↔ 2040-360mm:2
- Flush:109: 2020-500mm:2 ↔ 2040-360mm:2
- Flush:110: 2020-500mm:2 ↔ 2040-360mm:2
- Mate:564: 2040-360mm:2 ↔ 2020-corner-bracket:23
- Mate:565: 2040-360mm:2 ↔ 2020-corner-bracket:11
- Mate:567: 2040-360mm:2 ↔ 2020-corner-bracket:7
- Flush:111 (-10 mm): 2040-360mm:2
- Mate:569: 2020-corner-bracket:7
- Mate:570: 2020-corner-bracket:6
- Mate:571: 2040-360mm:2 ↔ 2020-corner-bracket:6
- Mate:575: 2020-500mm:4 ↔ 2020-350mm:12
- Flush:114: 2020-500mm:4 ↔ 2020-350mm:12
- Mate:577: 2020-350mm:12 ↔ 2020-corner-bracket:44
- Mate:581: 2020-350mm:12 ↔ 2020-corner-bracket:49
- Mate:583: 2020-500mm:4 ↔ 2020-corner-bracket:44
- Mate:585: 2020-500mm:3 ↔ 2020-corner-bracket:49
- Mate:587: 2020-350mm:12 ↔ 2020-corner-bracket:45
- Mate:591: 2020-500mm:3 ↔ 2020-corner-bracket:49
- Mate:596: 2020-500mm:4 ↔ 2020-corner-bracket:44
- Mate:597: 2020-350mm:12 ↔ 2020-corner-bracket:45
- Mate:598: SH8:2 ↔ 2020-350mm:4
- Mate:599: SH8:2 ↔ 2020-350mm:4
- Mate:600: SH8:2 ↔ rod-8mm:1
- Mate:601: SH8:1 ↔ 2020-350mm:4
- Mate:602: SH8:1 ↔ 2020-350mm:4
- Mate:603: SH8:1 ↔ rod-8mm:2
- Mate:604 (20 mm): SH8:1 ↔ holder-bearing-z-axis:1
- Mate:605 (20 mm): SH8:2 ↔ holder-bearing-z-axis:1
- Mate:606: SH8:3 ↔ 2040-350mm:1
- Mate:607: SH8:3 ↔ 2040-350mm:1
- Flush:115: 2020-500mm:3 ↔ 2040-360mm:2
- Mate:608: SH8:4 ↔ rod-8mm:2
- Mate:609: SH8:4 ↔ 2040-350mm:1
- Mate:610: SH8:4 ↔ 2040-350mm:1
- Mate:611: SH8:3 ↔ rod-8mm:1
- Mate:612: holder-LMF8LUU-z-axis-v2:1 ↔ LMF8LUU:1
- Mate:613: holder-LMF8LUU-z-axis-v2:1 ↔ LMF8LUU:1
- Mate:614: holder-LMF8LUU-z-axis-v2:1 ↔ LMF8LUU:1
- Mate:615: holder-LMF8LUU-z-axis-v2:1 ↔ 2020-240mm:1
- Mate:616: holder-LMF8LUU-z-axis-v2:1 ↔ 2020-240mm:1
- Mate:617: holder-LMF8LUU-z-axis-v2:2 ↔ 2020-240mm:1
- Mate:619: holder-LMF8LUU-z-axis-v2:2 ↔ 2020-240mm:1
- Mate:620: holder-LMF8LUU-z-axis-v2:2 ↔ LMF8LUU:2
- Mate:621: holder-LMF8LUU-z-axis-v2:2 ↔ LMF8LUU:2
- Mate:622: holder-LMF8LUU-z-axis-v2:2 ↔ LMF8LUU:2
- Mate:623: holder-LMF8LUU-z-axis-v2:1 ↔ 2020-240mm:1
